# Autodesk Inventor assembly: SR-042-DPY
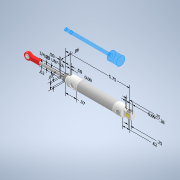
[picture p0: Inventor's stored thumbnail of the model, 180x180]
Saved by Autodesk Inventor 2022.3 (Build 263350000, 350)
## iProperties
Category: PARTsolutions
Company: BIMBA
Created: 2023-01-11
Part Number: SR-042-DPY
Catalog Web Link: www.cadenas.de
Description: Original Line Standard Air Cylinders-Standard Air Cylinders
Vendor: BIMBA
Document SubType Name: Assembly
Designer: psAdmin
Manufacturer: BIMBA
Mass: 31.591 g
Surface Area: 233.687 cm^2
Volume: 31.591 cm^3
Density: 1 g/cm^3
PSOL_IDENT_0: {$CADENAS_DATA/23d-libs/bimba/bimba_brand/bimba_imperial/bimba_full_line/original_line_cylinders/sta
PSOL_IDENT_1: ndard_air_cylinders/standard_air_cylinder_asmtab.prj},328 {VTYP=3D},{STYP=ASSTAB},{NB=SR-042-DPY},{L
PSOL_IDENT_2: INA=SR-042-DPY},{NN=Original Line Standard Air Cylinders},{DATE=23.12.2022 11:38:32},{GEOMDATE=21.09
PSOL_IDENT_3: .2022 06:44:35},{VERSION=},{LINEID=50},{WBVAR=STROKE,ACTING,MNT,DER,NR,BM,CO,OO,VO,M,EE,EEL,K,Q,Y,G,
PSOL_IDENT_4: T,HL,B,H,SER,SR,NT,W,STPT1,STPT2,STPT3,STPT4,MB,PB,PRC,TB,MN},{WBNUMERIC=STROKE,EEL}  {NB=SR-042-DPY
PSOL_IDENT_5: },{LINA=SR-042-DPY},{KT=DUMMY},{PN=SR-042-DPY},{PNC=SR-042-DPY},{PNA=(NO ACCESSORIES)},{PNAHELP=},{D
PSOL_IDENT_6: ASH=-},{BORE1=0.75000000},{BORE=3/4\" (04)},{BOREPN=04},{STROKE=2.000},{STROKEALG=[0.011:50/0.001]},
PSOL_IDENT_7: {STROKE1=2.000},{ACTING=D},{ACTINGALG= '' , 'Single Acting' , 'R' , 'Reverse Single Acting (R)' , 'D'
PSOL_IDENT_8: , 'Double Acting (D)' },{ACTINGPN=D},{MNT=P},{MNTALG= '' , 'Front Nose Mounting' , 'P' , 'Rear Pivo
PSOL_IDENT_9: t Mounting (P)' , 'XP' , 'Double End or Pivot Mounting (XP)' , 'X' , 'Double End Mounting (X)' , 'BF'
PSOL_IDENT_10: , 'Front Block Mounting (BF)' , 'BR' , 'Rear Block Mounting for Vertical Positioning (BR)' , 'BFT'
PSOL_IDENT_11: , 'Front Block Trunnion Mounting (BFT)' , 'BRT' , 'Rear Block Trunnion Mounting (BRT)' },{TYPE=SR-},
PSOL_IDENT_12: {MNTPN=P},{DER=},{DERALG= '' , 'N/A' },{NR=},{NRALG= '' , 'N/A' },{NRPN=},{BM=},{BMALG= '' , 'N/A' }
PSOL_IDENT_13: ,{BMPN=},{CO=},{COALG= '' , 'N/A' },{OO=},{OOALG= '', 'N/A' },{OOPN=},{VO=Z},{VOALG= 'Z' , 'N/A' },{
PSOL_IDENT_14: VOPN=},{OOVOPN=},{M=},{MALG= '', 'Without Magnet', 'M', 'With Magnet' },{EE=},{EEL=0.000},{EEMAX=48.
PSOL_IDENT_15: 0000},{EEALG= '', 'Without Extra Extension', 'EE', 'With Extra Extension' },{EELALG=0},{EEPN=},{EEPN
PSOL_IDENT_16: 1=0.000},{K=},{KALG= '', 'Standard' , 'K' , 'Ports Rotated 90deg K' },{KPN=},{Q=},{QALG= '' , 'N/A'
PSOL_IDENT_17: },{QPN=},{Y=Y},{YALG= '' , 'Without Pivot Bushing' , 'Y' , 'With Pivot Bushing' },{YPN=Y},{YCON=Y},{
PSOL_IDENT_18: F=},{FALG= '', 'Non-Coated (Standard)', 'F', 'Molycoated' },{FPN=},{G=},{GPN=},{GPN99=},{T=},{TALG= ''
PSOL_IDENT_19: , 'Standard -20° to 200°F (-29° to 95°C)' , 'N' , 'Low Temperature' , 'V' , 'High Temperature' },{N
PSOL_IDENT_20: PN=},{VPN=},{HL=},{HLALG= '' , 'Without Low Pressure Hydraulic' , 'HL' , 'With Low Pressure Hydrauli
PSOL_IDENT_21: c' },{B=},{BALG= '', 'W/out Bumpers' , 'B' , 'W/ Bumpers' },{BPN=},{H=},{HALG= '', 'N/A' },{HPN=},{S
PSOL_IDENT_22: ER=},{SERALG= '' , 'Without Spring Extend/Return' , 'JS' , 'With Spring Return' , 'JR' , 'With Sprin
PSOL_IDENT_23: g Extend' },{SR=SR},{SRALG= 'C' , 'Standard Blackened Carbon Steel' , 'SR' , 'Stainless Steel [SR]'
PSOL_IDENT_24: },{SRPN=SR},{SRCON=1},{NT=},{NTPN=},{W=},{WALG= '' , 'Without Wiper' , 'W' , 'With Wiper' },{WPN=},{
PSOL_IDENT_25: E=},{EALG= '' , 'Standard Seals/Lube' , 'E' , 'Non-Lube Seals/Lube' },{EPN=},{ST=},{STALG= '' , 'N/A'
PSOL_IDENT_26: },{STPT1=},{STPT1ALG= '' , 'N/A' },{STPT2=},{STPT2ALG= '' , 'N/A' },{STPT3=},{STPT3ALG= '' , 'N/A'
PSOL_IDENT_27: },{STPT4=},{STPT4ALG= '' , 'N/A' },{STPN=},{MB=},{MBALG= '' , 'N/A' },{MBPN=},{MBPNALL=},{MBPNALLREA
PSOL_IDENT_28: R=},{PB=},{PBALG= '' , 'Without Pivot Bracket' , 'D-13498-A' , 'D-13498-A' },{PBPN=},{PBPNALL=D-1349
PSOL_IDENT_29: 8-A},{PRC=},{PRCALG= '' , 'W/out Pivot Rod Clevis' , 'F,D-166-3' , 'D-166-3 (front)' },{PRCPN=},{PRC
PSOL_IDENT_30: PNALL=D-166-3},{TB=},{TBALG= '' , 'N/A' },{TBPN=},{TBPNALL=},{MN=},{MNALG= '' , 'Without Mounting Nu
PSOL_IDENT_31: t' , 'F,D-9' , 'D-9 (front)' , 'R,D-9' , 'D-9 (rear)', '2x,D-9' , 'D-9 (front & rear)' },{MNPN=},{MN
PSOL_IDENT_32: CONF=},{MNCONR=},{TLEN=3.2555},{FRAC=8.7500},{RGCON=},{RGDACCON=R},{RHCON=P},{RHCON1=P},{RHCONON=1},
PSOL_IDENT_33: {RHACCON=},{FNUTCON=0},{RNUTCON=0},{FNUTPN=D-9},{RNUTPN=D-9},{FNUTTRANS=0.0000},{RNUTTRANS=0.0000},{
PSOL_IDENT_34: VHOLECON=0},{A1=1.5940},{A1N=0.8750},{A1P=1.5940},{A1B=1.5940},{A4=0.2525},{A4N=0.3130},{A4P=0.2525}
PSOL_IDENT_35: ,{A5=0.0300},{A1H=1.594},{A1NH=0.5310},{A1PH=1.5940},{A1BH=1.0940},{A1SH=1.2190},{A2H=0.2190},{A2NH=
PSOL_IDENT_36: 0.2190},{LENGTH=3.7500},{LENGTH1=3.7500},{LENGTH2=3.8100},{MUL=2.0000},{MUL11=2.0000},{MUL22=5.38},{
PSOL_IDENT_37: MUL33=3.3800},{MUL2=2.0000},{MUL211=2.0000},{MUL222=2.6900},{MUL233=1.6900},{SSS=4.0000},{RGLEN=1.37
PSOL_IDENT_38: 15},{RHLEN=1.1230},{SSS1=3.0000},{A13=1.3120},{DIF=0.0000},{G5=0.6250},{ON=0},{SSADD=0.0000},{BADD=0
PSOL_IDENT_39: .0000},{MADD=0.0000},{NVADD=0.0000},{TRACKL=2.9655},{TRACKCON=D-74168},{TRIMCON=0},{TRIMCON1=0},{PIN
PSOL_IDENT_40: CON=D-51},{FSPACE=0.5448},{SPACE=0.0643},{TEXT=0.1125},{S1=1.0000},{D1=0.8325},{D1N=0.8050},{D1B=0.8
PSOL_IDENT_41: 625},{D1P=0.8325},{FA=0.940},{RA=0.9400},{PPATH=standard_air_cylinder_asmtpl.prj},{MATALGHTML=<b>Sta
PSOL_IDENT_42: ndard Original Line:</b><dl><dt>Rod:</dt><dd>- Stainless Steel</dd><dd>&nbsp;&nbsp;(5/16 9/16 Bores)
PSOL_IDENT_43: </dd><dd>- High Strength Carbon Steel</dd><dd>&nbsp;&nbsp;(3/4 3 Bore)</dd><dd>- Stainless Steel</dd
PSOL_IDENT_44: ><dd>&nbsp;&nbsp;(X style DXP/DX/DXDE)</dd><dt>Bearings:</dt><dd>- Sintered Bronze</dd><dt>Body:</dt
PSOL_IDENT_45: ><dd>- 304 Stainless Steel</dd><dt>End Caps:</dt><dd>- Aluminum</dd><dt>Seals:</dt><dd>- Buna N</dd>
PSOL_IDENT_46: </dl>},{ASSCFGPRA=04DP},{MBPNA=},{MNPNA=},{PRCPNA=},{ASSOPTACC=STPT4},{A=5.75},{HADD=0.0000},{WFL=0.
PSOL_IDENT_47: 25},{QADD=0.000},{QADD1=0.440},{TEST=2.0000},{MNTB=},{STDNUTF=0},{STDNUTR=0},{STRK2D=0},{X2D=2},{STR
PSOL_IDENT_48: OKESW=2.000},{EESW=0.000},{FCD=0},{BCD=0},{RCD=0},{CUSTADD=1.000},{FT=1/4-28 UNF-2A},{FT1=1/4-28 UNF
PSOL_IDENT_49: -2A},{FT2=5/8-18 UNF-2A},{PORT=1/8 NPT},{PORT1=1/8 NPT},{PORT2=1/8 NPT},{FT11=1/2-20 UNF-2A},{FT12=5
PSOL_IDENT_50: /8-18 UNF-2A},{B1=}
NB: SR-042-DPY
NN: Original Line Standard Air Cylinders
NT: Threaded (Standard)
NBSYN: $PNC.
LINA: SR-042-DPY
CATALOG: Bimba Products
PN: SR-042-DPY
PNA: (NO ACCESSORIES)
BORE: 3/4" (04)
STROKE: 2
ACTING: Double Acting (D)
MNT: Rear Pivot Mounting (P)
DER: N/A
NR: N/A
CO: N/A
OO: N/A
VO: N/A
M: Without Magnet
EE: Without Extra Extension
EEL: 0
K: Standard
Q: N/A
Y: With Pivot Bushing
G: Standard Lube
T: Standard -20° to 200°F (-29° to 95°C)
HL: Without Low Pressure Hydraulic
B: W/out Bumpers
H: N/A
SER: Without Spring Extend/Return
SR: Stainless Steel [SR]
W: Without Wiper
STPT1: N/A
STPT2: N/A
STPT3: N/A
STPT4: N/A
MB: N/A
PB: Without Pivot Bracket
PRC: W/out Pivot Rod Clevis
TB: N/A
MN: Without Mounting Nut
A: 5.75
SUPPLIER: BIMBA
ARTICLENO: SR-042-DPY
BOMINFO: SR-042-DPY
CREATOR: CADENAS GmbH
Title: SR-042-DPY
Author: Cadenas PARTsolutions
Comments: Standard Air Cylinders
## Documents named in this file (8)
- C:\Users\mavericks\Desktop\2023-Charged-Up\COMMON PARTS\AIR CYLINDERS\BIMBA_SR042DPY\AIS2022\SR-042-DPY.iam
- C:\Users\mavericks\Desktop\2023-Charged-Up\COMMON PARTS\AIR CYLINDERS\BIMBA_SR042DPY\AIS2022\SR-042-DPSRY0000000_0_dummy.ipt
- C:\Users\mavericks\Desktop\2023-Charged-Up\COMMON PARTS\AIR CYLINDERS\BIMBA_SR042DPY\AIS2022\04R000-0_rod_guide.ipt
- C:\Users\mavericks\Desktop\2023-Charged-Up\COMMON PARTS\AIR CYLINDERS\BIMBA_SR042DPY\AIS2022\04R-3_25550SR.ipt
- C:\Users\mavericks\Desktop\2023-Charged-Up\COMMON PARTS\AIR CYLINDERS\BIMBA_SR042DPY\AIS2022\04P0Y000_rear_head.ipt
- C:\Users\mavericks\Desktop\2023-Charged-Up\COMMON PARTS\AIR CYLINDERS\BIMBA_SR042DPY\AIS2022\D-3543.ipt
- C:\Users\mavericks\Desktop\2023-Charged-Up\COMMON PARTS\AIR CYLINDERS\BIMBA_SR042DPY\AIS2022\SR-042-DPY0000_rod.ipt
- C:\Users\mavericks\Desktop\2023-Charged-Up\COMMON PARTS\AIR CYLINDERS\TieRod End\60685K311_PTFE-LINED ALUMINUM BALL JOINT ROD END.ipt
## Components (7 placed, 7 different names)
1. SR-042-DPSRY0000000_0_dummy:1
2. 04R000-0_rod_guide:1 — Insert:1
3. 04R-3_25550SR:1
4. 04P0Y000_rear_head:1 — Angle:1
5. D-3543:1
6. SR-042-DPY0000_rod:1 — Insert:1, Insert:2
7. 60685K311_PTFE-LINED ALUMINUM BALL JOINT ROD END:1 — Insert:2, Angle:1
## Relationships (3: Insert 2, Angle 1)
- Insert:1: 04R000-0_rod_guide:1 ↔ SR-042-DPY0000_rod:1
- Insert:2 (6.35 mm): SR-042-DPY0000_rod:1 ↔ 60685K311_PTFE-LINED ALUMINUM BALL JOINT ROD END:1
- Angle:1 (0 deg): 04P0Y000_rear_head:1 ↔ 60685K311_PTFE-LINED ALUMINUM BALL JOINT ROD END:1
